# Autodesk Inventor assembly: undergroundPipe
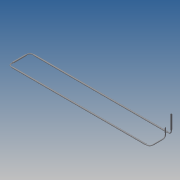
[picture p0: Inventor's stored thumbnail of the model, 180x180]
Saved by Autodesk Inventor 2014 SP1 (Build 180222100, 222)
## iProperties
Created: 2014-05-20
Part Number: undergroundPipe
Document SubType Name: Assembly
Designer: Dave
Author: Dave
## Documents named in this file (6)
- C:\Users\Dave\Desktop\hera-cad\Node\undergroundPipe.iam
- C:\Users\Dave\Desktop\hera-cad\Node\sweep.ipt
- C:\Users\Dave\Desktop\hera-cad\Node\pipe12m.ipt
- C:\Users\Dave\Desktop\hera-cad\Node\pipe1.5m.ipt
- C:\Users\Dave\Desktop\hera-cad\Node\pipe0.5m.ipt
- C:\Users\Dave\Desktop\hera-cad\Node\pipe0.85m.ipt
## Components (11 placed, 5 different names)
1. pipe12m:1 — Insert:1, Insert:2
2. sweep:1 — Insert:1, Insert:12
3. sweep:2 — Insert:2, Insert:3
4. sweep:4 — Insert:4, Insert:5
5. pipe1.5m:1 — Insert:3, Insert:4
6. pipe12m:2 — Insert:5, Insert:14
7. sweep:5 — Insert:14, Insert:15
8. sweep:6 — Insert:13, Insert:16
9. pipe0.5m:3 — Insert:13
10. pipe1.5m:2 — Insert:12
11. pipe0.85m:1 — Insert:15, Insert:16
## Relationships (10: Insert 10)
- Insert:1: pipe12m:1 ↔ sweep:1
- Insert:2: pipe12m:1 ↔ sweep:2
- Insert:3: sweep:2 ↔ pipe1.5m:1
- Insert:4: sweep:4 ↔ pipe1.5m:1
- Insert:5: sweep:4 ↔ pipe12m:2
- Insert:12: sweep:1 ↔ pipe1.5m:2
- Insert:13: sweep:6 ↔ pipe0.5m:3
- Insert:14: pipe12m:2 ↔ sweep:5
- Insert:15: sweep:5 ↔ pipe0.85m:1
- Insert:16: sweep:6 ↔ pipe0.85m:1
